# Autodesk Inventor assembly: all together
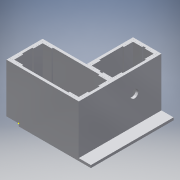
[picture p0: Inventor's stored thumbnail of the model, 180x180]
Saved by Autodesk Inventor 2016 (Build 200138000, 138)
## iProperties
Created: 2017-03-30
Part Number: all together
Document SubType Name: Assembly
Designer: Ethan
Mass: 3023.33 g
Surface Area: 4371.9 cm^2
Volume: 1119.75 cm^3
Density: 2.7 g/cm^3
Author: Ethan
## Documents named in this file (10)
- F:\RSX structure separate walls\all together.iam
- F:\RSX structure separate walls\wall 1.ipt
- F:\RSX structure separate walls\wall 2.ipt
- F:\RSX structure separate walls\wall 3.ipt
- F:\RSX structure separate walls\wall 4.ipt
- F:\RSX structure separate walls\wall 6.ipt
- F:\RSX structure separate walls\wall 5.ipt
- F:\RSX structure separate walls\wall braket.ipt
- F:\RSX structure separate walls\RSX bottom.ipt
- F:\RSX structure separate walls\RSX top.ipt
## Components (16 placed, 9 different names)
1. wall 1:1 — Rigid:1, Rigid:4, Mate:2, Mate:6
2. wall 2:1 — Rigid:1, Rigid:2, Mate:5, Flush:3, Mate:7, Flush:4, Mate:11, Mate:15, Flush:8, Mate:21
3. wall 3:1 — Rigid:2, Rigid:3, Mate:13, Mate:16, Mate:18, Mate:20
4. wall 4:1 — Rigid:3, Mate:10, Flush:5, Mate:14, Flush:7
5. wall 6:1 — Rigid:4, Rigid:5, Mate:1, Flush:1, Mate:4
6. wall 5:1 — Rigid:5, Mate:3, Flush:2, Mate:8, Mate:9, Mate:12, Flush:6, Mate:17, Mate:19
7. wall braket:1 — Mate:7, Mate:8, Flush:4
8. wall braket:2 — Mate:5, Mate:6, Flush:3
9. wall braket:3 — Mate:3, Mate:4, Flush:2
10. wall braket:4 — Mate:1, Mate:2, Flush:1
11. wall braket:5 — Mate:9, Mate:10, Flush:5
12. wall braket:6 — Mate:13, Mate:14, Flush:7
13. wall braket:7 — Mate:15, Mate:16, Flush:8
14. wall braket:8 — Mate:11, Mate:12, Flush:6
15. RSX bottom:1 — Mate:17, Mate:18
16. RSX top:1 — Mate:19, Mate:20, Mate:21
## Relationships (34: Mate 21, Flush 8, WeldJoint 5)
- Rigid:1 [WeldJoint]: wall 1:1 ↔ wall 2:1
- Rigid:2 [WeldJoint]: wall 2:1 ↔ wall 3:1
- Rigid:3 [WeldJoint]: wall 3:1 ↔ wall 4:1
- Rigid:4 [WeldJoint]: wall 1:1 ↔ wall 6:1
- Rigid:5 [WeldJoint]: wall 6:1 ↔ wall 5:1
- Mate:1: wall 6:1 ↔ wall braket:4
- Mate:2: wall 1:1 ↔ wall braket:4
- Flush:1: wall 6:1 ↔ wall braket:4
- Mate:3: wall 5:1 ↔ wall braket:3
- Mate:4: wall 6:1 ↔ wall braket:3
- Flush:2: wall 5:1 ↔ wall braket:3
- Mate:5: wall 2:1 ↔ wall braket:2
- Mate:6: wall 1:1 ↔ wall braket:2
- Flush:3: wall 2:1 ↔ wall braket:2
- Mate:7: wall 2:1 ↔ wall braket:1
- Mate:8: wall 5:1 ↔ wall braket:1
- Flush:4: wall 2:1 ↔ wall braket:1
- Mate:9: wall 5:1 ↔ wall braket:5
- Mate:10: wall 4:1 ↔ wall braket:5
- Flush:5: wall 4:1 ↔ wall braket:5
- Mate:11: wall 2:1 ↔ wall braket:8
- Mate:12: wall 5:1 ↔ wall braket:8
- Flush:6: wall 5:1 ↔ wall braket:8
- Mate:13: wall 3:1 ↔ wall braket:6
- Mate:14: wall 4:1 ↔ wall braket:6
- Flush:7: wall 4:1 ↔ wall braket:6
- Mate:15: wall 2:1 ↔ wall braket:7
- Mate:16: wall 3:1 ↔ wall braket:7
- Flush:8: wall 2:1 ↔ wall braket:7
- Mate:17: wall 5:1 ↔ RSX bottom:1
- Mate:18: wall 3:1 ↔ RSX bottom:1
- Mate:19: wall 5:1 ↔ RSX top:1
- Mate:20 (12.7 mm): wall 3:1 ↔ RSX top:1
- Mate:21 (12.7 mm): wall 2:1 ↔ RSX top:1
